# Autodesk Inventor assembly: DTConnetor-8020
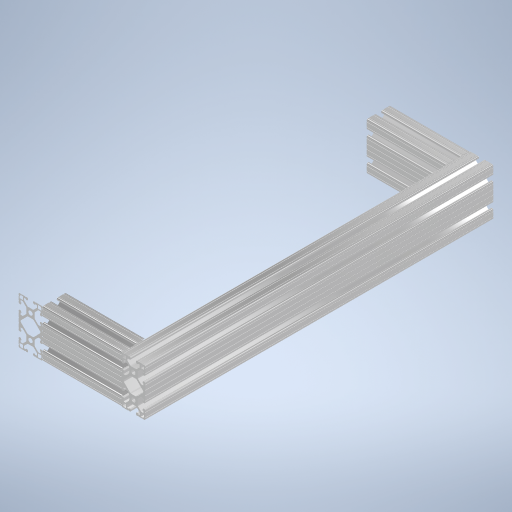
[picture p0: Inventor's stored thumbnail of the model, 512x512]
Saved by Autodesk Inventor 2023 (Build 270158000, 158)
## iProperties
Created: 2022-09-21
Part Number: DTConnetor-8020
Document SubType Name: Assembly
Designer: seene
Author: seene
## Documents named in this file (3)
- C:\Users\seene\Desktop\Stony Brook\SBRT\RoboRescue\Chassis\Frame\DTConnetor-8020.iam
- C:\Users\seene\Desktop\Stony Brook\SBRT\RoboRescue\Chassis\Frame\DTConnector-8020Length.ipt
- C:\Users\seene\Desktop\Stony Brook\SBRT\RoboRescue\Chassis\Frame\DTConnector-8020Width.ipt
## Components (4 placed, 2 different names)
1. DTConnector-8020Length:1 — Mate:3, Flush:5, Flush:6
2. DTConnector-8020Length:2 — Mate:1, Flush:1, Flush:2, Mate:2, Flush:3, Flush:4, Flush:5, Flush:6
3. DTConnector-8020Width:1 — Mate:2, Flush:3, Flush:4
4. DTConnector-8020Width:2 — Mate:1, Flush:1, Flush:2, Mate:3
## Relationships (9: Flush 6, Mate 3)
- Mate:1: DTConnector-8020Length:2 ↔ DTConnector-8020Width:2
- Flush:1: DTConnector-8020Length:2 ↔ DTConnector-8020Width:2
- Flush:2: DTConnector-8020Length:2 ↔ DTConnector-8020Width:2
- Mate:2: DTConnector-8020Length:2 ↔ DTConnector-8020Width:1
- Flush:3: DTConnector-8020Length:2 ↔ DTConnector-8020Width:1
- Flush:4: DTConnector-8020Length:2 ↔ DTConnector-8020Width:1
- Mate:3: DTConnector-8020Length:1 ↔ DTConnector-8020Width:2
- Flush:5: DTConnector-8020Length:1 ↔ DTConnector-8020Length:2
- Flush:6: DTConnector-8020Length:1 ↔ DTConnector-8020Length:2
